# Autodesk Inventor assembly: BG001_trajan20_22
(part 2 of 2)
- Passend:203 [Mate]: BT703_trajan20_21_Zeichenmaschine_v2_Plexi_Tür:1 ↔ AS 1427 - Metrisch M2 x 4:1
- Passend:204 [Mate]: BT703_trajan20_21_Zeichenmaschine_v2_Plexi_Tür:1 ↔ AS 1427 - Metrisch M2 x 4:2
- Passend:205 [Mate]: BT003_trajan20_22_Zeichenmaschine_neu_Fuß:1 ↔ BT201_trajan20_21_Zeichenmaschine_v2_Hauptplatte unten:1
- Passend:206 [Mate]: BT003_trajan20_22_Zeichenmaschine_neu_Fuß:1 ↔ BG000_trajan20_22_Zeichenmaschine_neu_Gestell:1
- Passend:207 [Mate]: BT003_trajan20_22_Zeichenmaschine_neu_Fuß:3 ↔ BT201_trajan20_21_Zeichenmaschine_v2_Hauptplatte unten:1
- Passend:208 [Mate]: BT003_trajan20_22_Zeichenmaschine_neu_Fuß:4 ↔ BT201_trajan20_21_Zeichenmaschine_v2_Hauptplatte unten:1
- Passend:209 [Mate]: BT003_trajan20_22_Zeichenmaschine_neu_Fuß:2 ↔ BT201_trajan20_21_Zeichenmaschine_v2_Hauptplatte unten:1
- Passend:210 [Mate]: BT003_trajan20_22_Zeichenmaschine_neu_Fuß:3 ↔ BG000_trajan20_22_Zeichenmaschine_neu_Gestell:1
- Passend:211 [Mate]: BT003_trajan20_22_Zeichenmaschine_neu_Fuß:2 ↔ BG000_trajan20_22_Zeichenmaschine_neu_Gestell:1
- Passend:212 [Mate]: BT003_trajan20_22_Zeichenmaschine_neu_Fuß:4 ↔ BG000_trajan20_22_Zeichenmaschine_neu_Gestell:1
- Passend:213 [Mate]: BT003_trajan20_22_Zeichenmaschine_neu_Fuß:6 ↔ BT202_trajan20_21_Zeichenmaschine_v2_getriebemotor platte unten:1
- Passend:214 [Mate]: BT003_trajan20_22_Zeichenmaschine_neu_Fuß:5 ↔ BT202_trajan20_21_Zeichenmaschine_v2_getriebemotor platte unten:1
- Passend:215 [Mate]: BT003_trajan20_22_Zeichenmaschine_neu_Fuß:6 ↔ BG000_trajan20_22_Zeichenmaschine_neu_Gestell:1
- Passend:216 [Mate]: BT003_trajan20_22_Zeichenmaschine_neu_Fuß:5 ↔ BG000_trajan20_22_Zeichenmaschine_neu_Gestell:1
- Passend:217 [Mate]: BG000_trajan20_22_Zeichenmaschine_neu_Gestell:1 ↔ BT706_trajan20_21_Zeichenmaschine_v2_Plexi_Haupt_Nothalt:1
- Fluchtend:14 [Flush]: BG000_trajan20_22_Zeichenmaschine_neu_Gestell:1 ↔ BT706_trajan20_21_Zeichenmaschine_v2_Plexi_Haupt_Nothalt:1
- Fluchtend:15 [Flush]: BG000_trajan20_22_Zeichenmaschine_neu_Gestell:1 ↔ BT706_trajan20_21_Zeichenmaschine_v2_Plexi_Haupt_Nothalt:1
- Passend:218 [Mate]: BT201_trajan20_21_Zeichenmaschine_v2_Hauptplatte unten:1 ↔ BT801_trajan20_21_Zeichenmaschine_neu_Netzteil:1
- Passend:219 [Mate]: BG000_trajan20_22_Zeichenmaschine_neu_Gestell:1 ↔ BT801_trajan20_21_Zeichenmaschine_neu_Netzteil:1
- Passend:220 [Mate] (1 mm): BG000_trajan20_22_Zeichenmaschine_neu_Gestell:1 ↔ BT801_trajan20_21_Zeichenmaschine_neu_Netzteil:1
- Passend:221 [Mate] (0.55 mm): BG000_trajan20_22_Zeichenmaschine_neu_Gestell:1 ↔ M5_Nutenstein_096215:29
- Passend:222 [Mate] (0.55 mm): BG000_trajan20_22_Zeichenmaschine_neu_Gestell:1 ↔ M5_Nutenstein_096215:33
- Passend:223 [Mate] (0.55 mm): BG000_trajan20_22_Zeichenmaschine_neu_Gestell:1 ↔ M5_Nutenstein_096215:32
- Passend:224 [Mate] (0.55 mm): BG000_trajan20_22_Zeichenmaschine_neu_Gestell:1 ↔ M5_Nutenstein_096215:30
- Passend:225 [Mate] (0.55 mm): BG000_trajan20_22_Zeichenmaschine_neu_Gestell:1 ↔ M5_Nutenstein_096215:31
- Passend:226 [Mate] (0.55 mm): BG000_trajan20_22_Zeichenmaschine_neu_Gestell:1 ↔ M5_Nutenstein_096215:34
- Winkel:38 [Angle] (0 deg): BG000_trajan20_22_Zeichenmaschine_neu_Gestell:1 ↔ M5_Nutenstein_096215:33
- Winkel:39 [Angle] (0 deg): BG000_trajan20_22_Zeichenmaschine_neu_Gestell:1 ↔ M5_Nutenstein_096215:32
- Winkel:40 [Angle] (0 deg): BG000_trajan20_22_Zeichenmaschine_neu_Gestell:1 ↔ M5_Nutenstein_096215:30
- Winkel:41 [Angle] (0 deg): BG000_trajan20_22_Zeichenmaschine_neu_Gestell:1 ↔ M5_Nutenstein_096215:31
- Winkel:42 [Angle] (0 deg): BG000_trajan20_22_Zeichenmaschine_neu_Gestell:1 ↔ M5_Nutenstein_096215:29
- Winkel:43 [Angle] (0 deg): BG000_trajan20_22_Zeichenmaschine_neu_Gestell:1 ↔ M5_Nutenstein_096215:34
- Passend:227 [Mate]: BT706_trajan20_21_Zeichenmaschine_v2_Plexi_Haupt_Nothalt:1 ↔ M5_Nutenstein_096215:29
- Passend:228 [Mate]: BT706_trajan20_21_Zeichenmaschine_v2_Plexi_Haupt_Nothalt:1 ↔ M5_Nutenstein_096215:33
- Passend:229 [Mate]: BT706_trajan20_21_Zeichenmaschine_v2_Plexi_Haupt_Nothalt:1 ↔ M5_Nutenstein_096215:32
- Passend:230 [Mate]: BT706_trajan20_21_Zeichenmaschine_v2_Plexi_Haupt_Nothalt:1 ↔ M5_Nutenstein_096215:34
- Passend:231 [Mate]: BT706_trajan20_21_Zeichenmaschine_v2_Plexi_Haupt_Nothalt:1 ↔ M5_Nutenstein_096215:30
- Passend:232 [Mate]: BT706_trajan20_21_Zeichenmaschine_v2_Plexi_Haupt_Nothalt:1 ↔ M5_Nutenstein_096215:31
- Einfügen:28 [Insert]: BT706_trajan20_21_Zeichenmaschine_v2_Plexi_Haupt_Nothalt:1 ↔ DIN 7984 M5 x 8:18
- Einfügen:29 [Insert]: BT706_trajan20_21_Zeichenmaschine_v2_Plexi_Haupt_Nothalt:1 ↔ DIN 7984 M5 x 8:19
- Einfügen:30 [Insert]: BT706_trajan20_21_Zeichenmaschine_v2_Plexi_Haupt_Nothalt:1 ↔ DIN 7984 M5 x 8:20
- Einfügen:31 [Insert]: BT706_trajan20_21_Zeichenmaschine_v2_Plexi_Haupt_Nothalt:1 ↔ DIN 7984 M5 x 8:21
- Einfügen:32 [Insert]: BT706_trajan20_21_Zeichenmaschine_v2_Plexi_Haupt_Nothalt:1 ↔ DIN 7984 M5 x 8:22
- Einfügen:33 [Insert]: BT706_trajan20_21_Zeichenmaschine_v2_Plexi_Haupt_Nothalt:1 ↔ DIN 7984 M5 x 8:23
- Passend:233 [Mate] (50 mm): BT201_trajan20_21_Zeichenmaschine_v2_Hauptplatte unten:1 ↔ Zeichenmaschine:1
- Passend:235 [Mate]: BG000_trajan20_22_Zeichenmaschine_neu_Gestell:1 ↔ Zeichenmaschine:1
- Passend:236 [Mate]: BT706_trajan20_21_Zeichenmaschine_v2_Plexi_Haupt_Nothalt:1 ↔ baugruppe:1
- Passend:237 [Mate] (0.1 mm): BT706_trajan20_21_Zeichenmaschine_v2_Plexi_Haupt_Nothalt:1 ↔ baugruppe:1
- Passend:239 [Mate]: BT706_trajan20_21_Zeichenmaschine_v2_Plexi_Haupt_Nothalt:1 ↔ Type-C Ext CBL - FEMALE +conn:1
- Passend:240 [Mate] (0.1 mm): BT706_trajan20_21_Zeichenmaschine_v2_Plexi_Haupt_Nothalt:1 ↔ Type-C Ext CBL - FEMALE +conn:1
- Passend:241 [Mate] (0.1 mm): BT706_trajan20_21_Zeichenmaschine_v2_Plexi_Haupt_Nothalt:1 ↔ Type-C Ext CBL - FEMALE +conn:1
- Passend:242 [Mate]: baugruppe:1 ↔ AS 1427 - Metrisch M3 x 5:1
- Passend:243 [Mate]: baugruppe:1 ↔ AS 1427 - Metrisch M3 x 5:2
- Passend:244 [Mate] (0.1 mm): BT706_trajan20_21_Zeichenmaschine_v2_Plexi_Haupt_Nothalt:1 ↔ baugruppe:1
- Einfügen:34 [Insert]: Type-C Ext CBL - FEMALE +conn:1 ↔ CNS 9671 M3 x 10:1
- Einfügen:35 [Insert]: Type-C Ext CBL - FEMALE +conn:1 ↔ CNS 9671 M3 x 10:2
- Passend:245 [Mate] (2 mm): BG000_trajan20_22_Zeichenmaschine_neu_Gestell:1 ↔ Zeichenmaschine:1
- Passend:246 [Mate]: BT102_trajan20_21_Zeichenmaschine_v2_Platte Getriebemotor:2 ↔ M5_Nutenstein_096215:7
- Passend:247 [Mate]: BT102_trajan20_21_Zeichenmaschine_v2_Platte Getriebemotor:2 ↔ M5_Nutenstein_096215:7
- Passend:248 [Mate]: BT102_trajan20_21_Zeichenmaschine_v2_Platte Getriebemotor:2 ↔ Senkschraube DIN 965 M5x14 51305_050_014(High):9
- Passend:249 [Mate]: Schraube ISO 14583:2011(E) M2,5x5-4.8:1 ↔ BT102_trajan20_21_Zeichenmaschine_v2_Platte Getriebemotor:2
- Passend:250 [Mate]: Schraube ISO 14583:2011(E) M2,5x5-4.8:4 ↔ BT102_trajan20_21_Zeichenmaschine_v2_Platte Getriebemotor:2
- Passend:251 [Mate]: Schraube ISO 14583:2011(E) M2,5x5-4.8:3 ↔ BT102_trajan20_21_Zeichenmaschine_v2_Platte Getriebemotor:2
- Passend:252 [Mate]: Schraube ISO 14583:2011(E) M2,5x5-4.8:2 ↔ BT102_trajan20_21_Zeichenmaschine_v2_Platte Getriebemotor:2
- Passend:253 [Mate]: Schraube ISO 14583:2011(E) M2,5x5-4.8:1 ↔ BT102_trajan20_21_Zeichenmaschine_v2_Platte Getriebemotor:2
- Einfügen:36 [Insert]: Schraube ISO 14583:2011(E) M2,5x8-4.8:1 ↔ BT101_trajan20_21_Zeichenmaschine_v2_Platte Stepper Motoren:2
- Einfügen:37 [Insert]: Schraube ISO 14583:2011(E) M2,5x8-4.8:2 ↔ BT101_trajan20_21_Zeichenmaschine_v2_Platte Stepper Motoren:2
- Einfügen:38 [Insert]: Schraube ISO 14583:2011(E) M2,5x8-4.8:3 ↔ BT101_trajan20_21_Zeichenmaschine_v2_Platte Stepper Motoren:2
- Einfügen:39 [Insert]: Schraube ISO 14583:2011(E) M2,5x8-4.8:4 ↔ BT101_trajan20_21_Zeichenmaschine_v2_Platte Stepper Motoren:2
- Einfügen:40 [Insert]: Schraube ISO 14583:2011(E) M2,5x8-4.8:5 ↔ BT101_trajan20_21_Zeichenmaschine_v2_Platte Stepper Motoren:2
- Einfügen:41 [Insert]: Schraube ISO 14583:2011(E) M2,5x8-4.8:8 ↔ BT101_trajan20_21_Zeichenmaschine_v2_Platte Stepper Motoren:2
- Einfügen:42 [Insert]: Schraube ISO 14583:2011(E) M2,5x8-4.8:7 ↔ BT101_trajan20_21_Zeichenmaschine_v2_Platte Stepper Motoren:2
- Einfügen:43 [Insert]: Schraube ISO 14583:2011(E) M2,5x8-4.8:6 ↔ BT101_trajan20_21_Zeichenmaschine_v2_Platte Stepper Motoren:2
- Passend:254 [Mate]: Steppermotor_NEMA17_17HS19-2004S1_Stepperonline:2 ↔ Schraube ISO 14583:2011(E) M2,5x8-4.8:5
- Passend:255 [Mate]: Steppermotor_NEMA17_17HS19-2004S1_Stepperonline:2 ↔ Schraube ISO 14583:2011(E) M2,5x8-4.8:7
- Passend:256 [Mate]: Steppermotor_NEMA17_17HS19-2004S1_Stepperonline:1 ↔ Schraube ISO 14583:2011(E) M2,5x8-4.8:3
- Passend:257 [Mate]: Steppermotor_NEMA17_17HS19-2004S1_Stepperonline:1 ↔ Schraube ISO 14583:2011(E) M2,5x8-4.8:1
- Passend:258 [Mate]: BT901_goteln20_23_Zeichenmaschine_stepper_getriebe_halterung:1 ↔ BT202_trajan20_21_Zeichenmaschine_v2_getriebemotor platte unten:1
- Passend:259 [Mate]: BT901_goteln20_23_Zeichenmaschine_stepper_getriebe_halterung:1 ↔ BT102_trajan20_21_Zeichenmaschine_v2_Platte Getriebemotor:2
- Passend:260 [Mate]: Schraube ISO 14583:2011(E) M3x12-4.8:2 ↔ BT202_trajan20_21_Zeichenmaschine_v2_getriebemotor platte unten:1
- Passend:261 [Mate]: Schraube ISO 14583:2011(E) M3x12-4.8:1 ↔ BT202_trajan20_21_Zeichenmaschine_v2_getriebemotor platte unten:1
- Passend:262 [Mate]: BT901_goteln20_23_Zeichenmaschine_stepper_getriebe_halterung:1 ↔ Schraube ISO 14583:2011(E) M3x12-4.8:1
- Passend:263 [Mate]: BT901_goteln20_23_Zeichenmaschine_stepper_getriebe_halterung:1 ↔ Schraube ISO 14583:2011(E) M3x12-4.8:2
- Passend:264 [Mate]: BT202_trajan20_21_Zeichenmaschine_v2_getriebemotor platte unten:1
- Winkel:44 [Angle] (0 deg): BT202_trajan20_21_Zeichenmaschine_v2_getriebemotor platte unten:1
- Passend:265 [Mate]: Schraube ISO 14583:2011(E) M3x12-4.8:2
- Einfügen:44 [Insert]: BT901_goteln20_23_Zeichenmaschine_stepper_getriebe_halterung:1 ↔ Linsenschraube mit geschmiedetem Innensechskant - Metrisch M3 x 0.5 x 12:1
- Einfügen:45 [Insert]: BT901_goteln20_23_Zeichenmaschine_stepper_getriebe_halterung:1 ↔ Linsenschraube mit geschmiedetem Innensechskant - Metrisch M3 x 0.5 x 12:2
- Einfügen:46 [Insert]: BT901_goteln20_23_Zeichenmaschine_stepper_getriebe_halterung:1 ↔ Linsenschraube mit geschmiedetem Innensechskant - Metrisch M3 x 0.5 x 3:3
- Passend:270 [Mate]: BT902_goteln20_23_Zeichenmaschine_neu_stepper_getriebe_winkel:1 ↔ BT102_trajan20_21_Zeichenmaschine_v2_Platte Getriebemotor:2
- Passend:272 [Mate]: BT901_goteln20_23_Zeichenmaschine_stepper_getriebe_halterung:1 ↔ BT902_goteln20_23_Zeichenmaschine_neu_stepper_getriebe_winkel:1
- Passend:273 [Mate]: BT902_goteln20_23_Zeichenmaschine_neu_stepper_getriebe_winkel:2 ↔ BT102_trajan20_21_Zeichenmaschine_v2_Platte Getriebemotor:2
- Passend:275 [Mate]: BT901_goteln20_23_Zeichenmaschine_stepper_getriebe_halterung:1 ↔ BT902_goteln20_23_Zeichenmaschine_neu_stepper_getriebe_winkel:2
- Passend:277 [Mate]: Linsenschraube mit geschmiedetem Innensechskant - Metrisch M3 x 0.5 x 10:2 ↔ BT102_trajan20_21_Zeichenmaschine_v2_Platte Getriebemotor:2
- Passend:278 [Mate]: Linsenschraube mit geschmiedetem Innensechskant - Metrisch M3 x 0.5 x 10:1 ↔ BT102_trajan20_21_Zeichenmaschine_v2_Platte Getriebemotor:2
- Passend:280 [Mate]: BT901_goteln20_23_Zeichenmaschine_stepper_getriebe_halterung:1 ↔ Steppermotor_NEMA17_17HS19-2004S1_Stepperonline:3
- Passend:281 [Mate]: BT901_goteln20_23_Zeichenmaschine_stepper_getriebe_halterung:1 ↔ Schraube ISO 14583:2011(E) M2,5x10-4.8:1
- Passend:282 [Mate]: BT901_goteln20_23_Zeichenmaschine_stepper_getriebe_halterung:1 ↔ Schraube ISO 14583:2011(E) M2,5x10-4.8:1
- Passend:283 [Mate]: Steppermotor_NEMA17_17HS19-2004S1_Stepperonline:3 ↔ Schraube ISO 14583:2011(E) M2,5x10-4.8:1
- Passend:284 [Mate]: Steppermotor_NEMA17_17HS19-2004S1_Stepperonline:3 ↔ Schraube ISO 14583:2011(E) M2,5x10-4.8:3
- Passend:285 [Mate] (1.6 mm): BT901_goteln20_23_Zeichenmaschine_stepper_getriebe_halterung:1 ↔ Schraube ISO 14583:2011(E) M2,5x10-4.8:3
- Passend:286 [Mate]: BT901_goteln20_23_Zeichenmaschine_stepper_getriebe_halterung:1 ↔ Schraube ISO 14583:2011(E) M2,5x10-4.8:3
- Passend:287 [Mate]: BT901_goteln20_23_Zeichenmaschine_stepper_getriebe_halterung:1 ↔ Schraube ISO 14583:2011(E) M2,5x10-4.8:3
- Passend:288 [Mate]: BT901_goteln20_23_Zeichenmaschine_stepper_getriebe_halterung:1 ↔ Schraube ISO 14583:2011(E) M2,5x10-4.8:2
- Passend:289 [Mate]: BT901_goteln20_23_Zeichenmaschine_stepper_getriebe_halterung:1 ↔ Schraube ISO 14583:2011(E) M2,5x10-4.8:4
- Passend:290 [Mate]: Steppermotor_NEMA17_17HS19-2004S1_Stepperonline:3 ↔ Schraube ISO 14583:2011(E) M2,5x10-4.8:4
- Passend:291 [Mate]: Steppermotor_NEMA17_17HS19-2004S1_Stepperonline:3 ↔ Schraube ISO 14583:2011(E) M2,5x10-4.8:2
- Passend:292 [Mate] (1.6 mm): BT901_goteln20_23_Zeichenmaschine_stepper_getriebe_halterung:1 ↔ Schraube ISO 14583:2011(E) M2,5x10-4.8:4
- Passend:293 [Mate] (1.6 mm): BT901_goteln20_23_Zeichenmaschine_stepper_getriebe_halterung:1 ↔ Schraube ISO 14583:2011(E) M2,5x10-4.8:2
- Passend:294 [Mate]: BT803_goteln20_22_Zeichenmaschine_neu_getriebe:1 ↔ BT102_trajan20_21_Zeichenmaschine_v2_Platte Getriebemotor:2
- Passend:295 [Mate]: BT803_goteln20_22_Zeichenmaschine_neu_getriebe:1 ↔ Schraube ISO 14583:2011(E) M2,5x5-4.8:2
- Passend:296 [Mate]: BT803_goteln20_22_Zeichenmaschine_neu_getriebe:1 ↔ Schraube ISO 14583:2011(E) M2,5x5-4.8:1
- Passend:297 [Mate]: BT803_goteln20_22_Zeichenmaschine_neu_getriebe:1 ↔ BT102_trajan20_21_Zeichenmaschine_v2_Platte Getriebemotor:2
- Passend:298 [Mate]: BT803_goteln20_22_Zeichenmaschine_neu_getriebe:1 ↔ Schraube ISO 14583:2011(E) M2,5x5-4.8:4
- Passend:299 [Mate]: Schraube ISO 14583:2011(E) M2,5x5-4.8:3 ↔ BT102_trajan20_21_Zeichenmaschine_v2_Platte Getriebemotor:2
- Passend:300 [Mate]: Steppermotor_NEMA17_17HS19-2004S1_Stepperonline:3 ↔ BT803_goteln20_22_Zeichenmaschine_neu_getriebe:1
- Fluchtend:16 [Flush]: BT803_goteln20_22_Zeichenmaschine_neu_getriebe:1 ↔ BT804_goteln20_22_Zeichenmaschine_neu_getriebe_lagerung:1
- Fluchtend:17 [Flush]: BT803_goteln20_22_Zeichenmaschine_neu_getriebe:1 ↔ BT804_goteln20_22_Zeichenmaschine_neu_getriebe_lagerung:1
- Passend:301 [Mate]: BT803_goteln20_22_Zeichenmaschine_neu_getriebe:1 ↔ BT804_goteln20_22_Zeichenmaschine_neu_getriebe_lagerung:1
- Einfügen:47 [Insert]: BT804_goteln20_22_Zeichenmaschine_neu_getriebe_lagerung:1 ↔ DIN 625 SKF SKF 623:1
- Passend:302 [Mate]: DIN 625 SKF SKF 623:1 ↔ BT805_goteln20_22_Zeichenmaschine_neu_getriebe_welle_5zu2:1
- Passend:303 [Mate]: DIN 625 SKF SKF 623:1 ↔ BT805_goteln20_22_Zeichenmaschine_neu_getriebe_welle_5zu2:1
- Passend:304 [Mate]: Steppermotor_NEMA17_17HS19-2004S1_Stepperonline:3 ↔ BT805_goteln20_22_Zeichenmaschine_neu_getriebe_welle_5zu2:1
- Passend:305 [Mate]: Steppermotor_NEMA17_17HS19-2004S1_Stepperonline:3 ↔ BS 4168 : Teil 2 Innensechskantschrauben und Stiftschlüssel, metrische Ausführung - Spezifikation für Sechskant-Gewindestifte mit Kegelstumpf - Metrisch M3 x 2:1
- Passend:306 [Mate]: BT805_goteln20_22_Zeichenmaschine_neu_getriebe_welle_5zu2:1 ↔ BS 4168 : Teil 2 Innensechskantschrauben und Stiftschlüssel, metrische Ausführung - Spezifikation für Sechskant-Gewindestifte mit Kegelstumpf - Metrisch M3 x 2:1
- Passend:307 [Mate]: BT805_goteln20_22_Zeichenmaschine_neu_getriebe_welle_5zu2:1 ↔ BS 4168 : Teil 2 Innensechskantschrauben und Stiftschlüssel, metrische Ausführung - Spezifikation für Sechskant-Gewindestifte mit Kegelstumpf - Metrisch M2 x 3:1
- Passend:308 [Mate]: BT805_goteln20_22_Zeichenmaschine_neu_getriebe_welle_5zu2:1 ↔ BT805_goteln20_22_Zeichenmaschine_neu_getriebe_welle:1
- Fluchtend:18 [Flush]: BT805_goteln20_22_Zeichenmaschine_neu_getriebe_welle_5zu2:1 ↔ BT805_goteln20_22_Zeichenmaschine_neu_getriebe_welle:1
- Passend:309 [Mate] (1 mm): BS 4168 : Teil 2 Innensechskantschrauben und Stiftschlüssel, metrische Ausführung - Spezifikation für Sechskant-Gewindestifte mit Kegelstumpf - Metrisch M2 x 3:1 ↔ BT805_goteln20_22_Zeichenmaschine_neu_getriebe_welle:1
- Passend:310 [Mate]: BT902_goteln20_23_Zeichenmaschine_neu_stepper_getriebe_winkel:1 ↔ Linsenschraube mit geschmiedetem Innensechskant - Metrisch M3 x 0.5 x 10:1
- Passend:311 [Mate]: BT902_goteln20_23_Zeichenmaschine_neu_stepper_getriebe_winkel:2 ↔ Linsenschraube mit geschmiedetem Innensechskant - Metrisch M3 x 0.5 x 12:2
